# Autodesk Inventor assembly: ASY TRM 040 seal
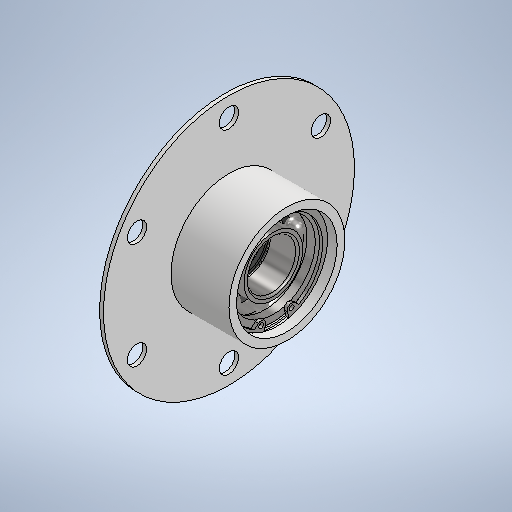
[picture p0: Inventor's stored thumbnail of the model, 512x512]
Saved by Autodesk Inventor 2025 (Build 290162010, 162A)
## iProperties
Created: 2024-09-08
Part Number: ASY TRM 040 seal
Document SubType Name: Assembly
Designer: pokla
Author: pokla
## Documents named in this file (6)
- C:\Users\pokla\Documents\Inventor\BSH_Beshkino_bio_tank\ASY TRM 040 seal.iam
- C:\Users\pokla\Documents\Inventor\BSH_Beshkino_bio_tank\TRM 041 flange.ipt
- C:\Users\pokla\Documents\Inventor\BSH_Beshkino_bio_tank\TRM 042 flange tube.ipt
- C:\Users\pokla\Documents\Inventor\Content Center Files\R2025\en-US\BS 290 SKF(02)\BS 290 SKF - SKF 7205 BE.ipt
- C:\Users\pokla\Documents\Inventor\Content Center Files\R2025\en-US\CSN 02 9401  G\CSN 02 9401 - G 25x52x7 - NBR.ipt
- C:\Users\pokla\Documents\Inventor\Content Center Files\R2025\en-US\ANSI B 27.7M(1)\ANSI B 27.7M - 3BMI-50.ipt
## Components (5 placed, 5 different names)
1. TRM 041 flange:1
2. TRM 042 flange tube:1
3. BS 290 SKF SKF 7205 BE:1
4. CSN 02 9401 G G 25x52x7 - NBR:1
5. ANSI B 27.7M 3BMI-50:1
## Relationships (5: WeldJoint 3, Mate 2)
- [WeldJoint]: TRM 041 flange:1 ↔ TRM 042 flange tube:1
- [WeldJoint]: TRM 041 flange:1 ↔ CSN 02 9401 G G 25x52x7 - NBR:1
- [WeldJoint] (-10 mm): TRM 041 flange:1 ↔ BS 290 SKF SKF 7205 BE:1
- [Mate]: TRM 042 flange tube:1 ↔ ANSI B 27.7M 3BMI-50:1
- [Mate]: TRM 042 flange tube:1 ↔ ANSI B 27.7M 3BMI-50:1
